# Autodesk Inventor assembly: rgb-controller-case
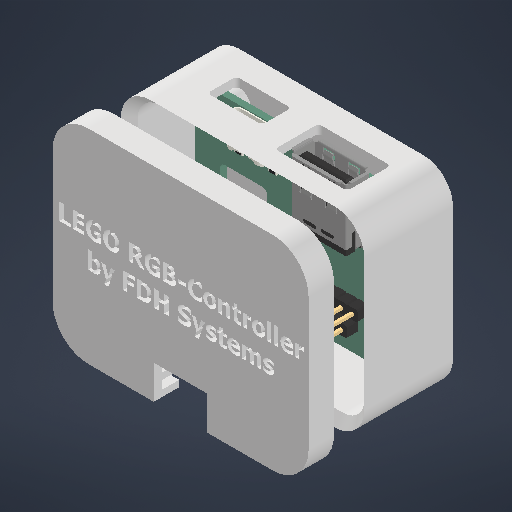
[picture p0: Inventor's stored thumbnail of the model, 512x512]
Saved by Autodesk Inventor 2026.2 (Build 302298000, 298)
## iProperties
Created: 2026-04-30
Part Number: rgb-controller-case
Document SubType Name: Assembly
Designer: FromDarkHell
Author: FromDarkHell
## iProperties of the stored document USB_C_Receptacle_GCT_USB4135-GF-A_6P_TopMnt_Horizontal.ipt
Created: 2026-04-30
Part Number: USB_C_Receptacle_GCT_USB4135-GF-A_6P_TopMnt_Horizontal
Material: Generic
Document SubType Name: Modeling
Designer: FromDarkHell
Density: 1 g/cm^3
Appearance: Default
Author: FromDarkHell
## iProperties of the stored document board-view.iam
Company: Kicad
Created: 2026-04-30
Part Number: board-view
Description: KiCad electronic assembly
Document SubType Name: Assembly
Designer: FromDarkHell
Authority: Unknown
Sending System: KiCad to STEP converter
Preprocessor: Open CASCADE STEP processor 7.9
Title: board-view.step
Author: Pcbnew
## iProperties of the stored document PinHeader_1x04_P2.54mm_Vertical.ipt
Created: 2026-04-30
Part Number: PinHeader_1x04_P2.54mm_Vertical
Material: Generic
Document SubType Name: Modeling
Designer: FromDarkHell
Density: 1 g/cm^3
Appearance: Default
Author: FromDarkHell
## iProperties of the stored document USB_A_Molex_67643_Horizontal.ipt
Created: 2026-04-30
Part Number: USB_A_Molex_67643_Horizontal
Material: Generic
Document SubType Name: Modeling
Designer: FromDarkHell
Density: 1 g/cm^3
Appearance: Default
Author: FromDarkHell
## iProperties of the stored document basic-rgb_PCB.ipt
Created: 2026-04-30
Part Number: basic-rgb_PCB
Material: Generic
Document SubType Name: Modeling
Designer: FromDarkHell
Density: 1 g/cm^3
Appearance: Default
Author: FromDarkHell
## iProperties of the stored document PinHeader_1x03_P2.54mm_Vertical.ipt
Created: 2026-04-30
Part Number: PinHeader_1x03_P2.54mm_Vertical
Material: Generic
Document SubType Name: Modeling
Designer: FromDarkHell
Density: 1 g/cm^3
Appearance: Default
Author: FromDarkHell
## iProperties of the stored document R_0805_2012Metric.ipt
Created: 2026-04-30
Part Number: R_0805_2012Metric
Material: Generic
Document SubType Name: Modeling
Designer: FromDarkHell
Density: 1 g/cm^3
Appearance: Default
Author: FromDarkHell
## Documents named in this file (11)
- J:\Coding Projecties\LegoDimensionsRGB\projects\rgb-controller\case\rgb-controller-case.iam
- **J:\Coding Projecties\LegoDimensionsRGB\projects\rgb-controller\case\rgb-controller-case.iam*LocalDocs*xAaaaaedaAaaaaaaaAaaaau1kPe*board-view.iam
- J:\Coding Projecties\LegoDimensionsRGB\projects\rgb-controller\case\BottomShell.ipt
- J:\Coding Projecties\LegoDimensionsRGB\projects\rgb-controller\case\TopShell.ipt
- **J:\Coding Projecties\LegoDimensionsRGB\projects\rgb-controller\case\rgb-controller-case.iam*LocalDocs*xAaaaamdaAaaaaaaaAaaaqmelJf*USB_C_Receptacle_GCT_USB4135-GF-A_6P_TopMnt_Horizontal.ipt
- **J:\Coding Projecties\LegoDimensionsRGB\projects\rgb-controller\case\rgb-controller-case.iam*LocalDocs*xAaaaqtaaAaaaaaaaAaaaacrtQf*PinHeader_1x03_P2.54mm_Vertical.ipt
- **J:\Coding Projecties\LegoDimensionsRGB\projects\rgb-controller\case\rgb-controller-case.iam*LocalDocs*xAaaaqtdaAaaaaaaaAaaaqangQd*R_0805_2012Metric.ipt
- **J:\Coding Projecties\LegoDimensionsRGB\projects\rgb-controller\case\rgb-controller-case.iam*LocalDocs*xAaaaavbaAaaaaaaaAaaaa4d44d*USB_A_Molex_67643_Horizontal.ipt
- **J:\Coding Projecties\LegoDimensionsRGB\projects\rgb-controller\case\rgb-controller-case.iam*LocalDocs*xAaaaqmbaAaaaaaaaAaaaani1Zf*PinHeader_1x04_P2.54mm_Vertical.ipt
- **J:\Coding Projecties\LegoDimensionsRGB\projects\rgb-controller\case\rgb-controller-case.iam*LocalDocs*xAaaaqtbaAaaaaaaaAaaaanwgUf*basic-rgb_PCB.ipt
- J:\Coding Projecties\LegoDimensionsRGB\projects\rgb-controller\schematic\board-view.step
## Components (3 placed, 3 different names)
1. board-view:1 [sub-assembly] — Mate:1, Mate:2
2. BottomShell:1 — Mate:1, Mate:2
3. TopShell:1
## Relationships (2: Mate 2)
- Mate:1: board-view:1 ↔ BottomShell:1
- Mate:2: board-view:1 ↔ BottomShell:1
